# Autodesk Inventor assembly: kvetinac_sestava
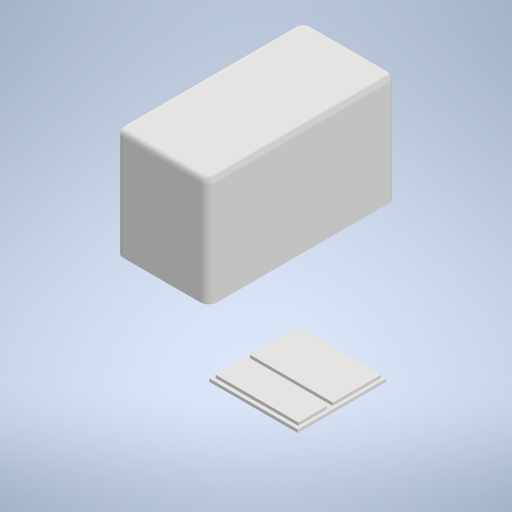
[picture p0: Inventor's stored thumbnail of the model, 512x512]
Saved by Autodesk Inventor 2024 (Build 280153000, 153)
## iProperties
Created: 2025-04-21
Part Number: kvetinac_sestava
Document SubType Name: Assembly
Designer: annav
Author: annav
## Documents named in this file (3)
- C:\Users\annav\Desktop\model\kvetinac_sestava.iam
- C:\Users\annav\Desktop\model\květináč.ipt
- C:\Users\annav\Desktop\model\víčko.ipt
## Components (2 placed, 2 different names)
1. květináč:1 — Proti sobě:1, Proti sobě:2, Proti sobě:3, Proti sobě:8, Proti sobě:9
2. víčko:1 — Proti sobě:8, Proti sobě:9
## Relationships (5: Mate 5)
- Proti sobě:1 [Mate]: květináč:1
- Proti sobě:2 [Mate]: květináč:1
- Proti sobě:3 [Mate]: květináč:1
- Proti sobě:8 [Mate]: květináč:1 ↔ víčko:1
- Proti sobě:9 [Mate]: květináč:1 ↔ víčko:1
